# Autodesk Inventor assembly: vehicle assembly v2
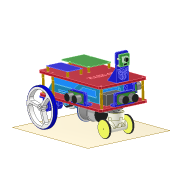
[picture p0: Inventor's stored thumbnail of the model, 180x180]
Saved by Autodesk Inventor 2022 (Build 260153000, 153)
## iProperties
Created: 2024-06-06
Part Number: vehicle assembly v2
Document SubType Name: Assembly
Designer: david
Author: david
## Documents named in this file (31)
- C:\Users\david\OneDrive\Documents\Inventor\WRO_FE_2024\vehicle assembly v2.iam
- C:\Users\david\OneDrive\Documents\Inventor\WRO_FE_2024\base plate.ipt
- C:\Users\david\OneDrive\Documents\Inventor\WRO_FE_2024\bearing holder.ipt
- C:\Users\david\OneDrive\Documents\Inventor\WRO_FE_2024\servo motor HS-7955TG.iam
- C:\Users\david\OneDrive\Documents\Inventor\WRO_FE_2024\steering.ipt
- C:\Users\david\OneDrive\Documents\Inventor\WRO_FE_2024\dfifferential.ipt
- C:\Users\david\OneDrive\Documents\Inventor\WRO_FE_2024\front wheel.ipt
- C:\Users\david\OneDrive\Documents\Inventor\WRO_FE_2024\driver gear.ipt
- C:\Users\david\OneDrive\Documents\Inventor\WRO_FE_2024\rear wheel 86mm.ipt
- C:\Users\david\OneDrive\Documents\Inventor\WRO_FE_2024\rear shaft v2.ipt
- rear shaft.ipt
- C:\Users\david\OneDrive\Documents\Inventor\WRO_FE_2024\12v DC motor mount.ipt
- C:\Users\david\OneDrive\Documents\Inventor\WRO_FE_2024\12v DC motor.ipt
- C:\Users\david\OneDrive\Documents\Inventor\WRO_FE_2024\driver gear adapter v2.ipt
- C:\Users\david\OneDrive\Documents\Inventor\WRO_FE_2024\stand M3-L10.ipt
- C:\Users\david\OneDrive\Documents\Inventor\WRO_FE_2024\top plate.ipt
- C:\Users\david\OneDrive\Documents\Inventor\WRO_FE_2024\raspberry pi.ipt
- C:\Users\david\OneDrive\Documents\Inventor\WRO_FE_2024\3s lipo battery.ipt
- C:\Users\david\OneDrive\Documents\Inventor\WRO_FE_2024\ultrasonic mount.ipt
- C:\Users\david\OneDrive\Documents\Inventor\WRO_FE_2024\US-015.ipt
- C:\Users\david\OneDrive\Documents\Inventor\WRO_FE_2024\stand M3-L30.ipt
- C:\Users\david\OneDrive\Documents\Inventor\WRO_FE_2024\LM2596 Buck Converter.ipt
- C:\Users\david\OneDrive\Documents\Inventor\WRO_FE_2024\camera mount.ipt
- C:\Users\david\OneDrive\Documents\Inventor\WRO_FE_2024\raspberry pi camera v2.ipt
- C:\Users\david\OneDrive\Documents\Inventor\WRO_FE_2024\stub.ipt
- C:\Users\david\OneDrive\Documents\Inventor\WRO_FE_2024\3S lipo holder.ipt
- C:\Users\david\OneDrive\Documents\Inventor\WRO_FE_2024\differential stopper.ipt
- C:\Users\david\OneDrive\Documents\Inventor\WRO_FE_2024\driver gear stopper.ipt
- C:\Users\david\OneDrive\Documents\Inventor\WRO_FE_2024\12v DC motor mount (3D printed).ipt
- C:\Users\david\OneDrive\Documents\Inventor\WRO_FE_2024\front shaft v3.ipt
- C:\Users\david\OneDrive\Documents\Inventor\WRO_FE_2024\steering bottom half.ipt
## Components (62 placed, 31 different names)
1. raspberry pi:2 — Insert:58, Insert:59
2. base plate:1 — Insert:60, Insert:61, Insert:62, Insert:63, Mate:9, Mate:10, Insert:72, Insert:73, Mate:11, Flush:6, Flush:7, Flush:8, Insert:74, Insert:75, Insert:128, Insert:129, Insert:130, Insert:131, Insert:132, Insert:133, Insert:134, Insert:135, Insert:136, Insert:137, Insert:138, Insert:139, Insert:140, Insert:141, Insert:144, Insert:145, Insert:154, Insert:155, Insert:156, Insert:157, Insert:158, Insert:159, Insert:160, Insert:161, Insert:162
3. top plate:1 — Insert:54, Insert:55, Insert:56, Insert:57, Insert:108, Insert:109, Insert:110, Insert:111, Insert:126, Insert:127, Insert:152, Insert:153
4. bearing holder:1 — Insert:138, Insert:139, Insert:142
5. bearing holder:2 — Insert:140, Insert:141
6. bearing holder:3 — Insert:136, Insert:137
7. bearing holder:4 — Insert:134, Insert:135, Insert:143
8. dfifferential:1
9. driver gear:1 — Insert:47
10. rear shaft v2: right — Insert:83, Angle:9, Insert:143
11. rear shaft v2: left — Insert:84, Angle:8, Insert:142
12. rear wheel 86mm: right — Insert:83, Angle:9
13. rear wheel 86mm: left — Tangent:1, Insert:84, Angle:8
14. 12v DC motor mount:1 — Insert:38, Insert:39, Insert:72, Insert:73
15. 12v DC motor:1 — Insert:38, Insert:39, Insert:46, Angle:5
16. driver gear adapter v2:1 — Insert:46, Insert:47, Angle:5
17. servo motor HS-7955TG:1 [sub-assembly] — Mate:2, Insert:20, Mate:9, Mate:10, Mate:11
18. steering:1 — Insert:20, Steering Angle, Insert:163, Insert:166, Insert:167
19. front wheel:1 — Insert:164, Angle:10
20. front wheel:2 — Insert:165, Angle:11
21. stand M3-L30:2 — Insert:60, Insert:150
22. stand M3-L30:3 — Insert:63, Insert:146
23. stand M3-L30:1 — Insert:61, Insert:151
24. stand M3-L30:4 — Insert:62, Insert:148
25. stand M3-L30:9 — Insert:74, Insert:149
26. stand M3-L30:10 — Insert:75, Insert:147
27. stand M3-L10:1 — Insert:55
28. stand M3-L10:2 — Insert:57
29. stand M3-L10:3 — Insert:54, Insert:59
30. stand M3-L10:4 — Insert:56, Insert:58
31. 3s lipo battery:1 — Mate:12, Mate:13, Flush:9
32. ultrasonic mount:1 — Insert:102, Insert:103, Insert:128, Insert:129
33. US-015:1 — Insert:102, Insert:103
34. ultrasonic mount:2 — Insert:104, Insert:105, Insert:130, Insert:131
35. ultrasonic mount:3 — Insert:106, Insert:107, Insert:132, Insert:133
36. US-015:2 — Insert:106, Insert:107
37. US-015:3 — Insert:104, Insert:105
38. LM2596 Buck Converter:1 — Insert:112, Insert:113
39. stand M3-L10:5 — Insert:109
40. stand M3-L10:6 — Insert:111
41. stand M3-L10:7 — Insert:108, Insert:112
42. stand M3-L10:8 — Insert:110, Insert:113
43. camera mount:1 — Insert:124, Insert:125, Insert:126, Insert:127
44. raspberry pi camera v2:1 — Insert:120, Insert:121, Insert:122, Insert:123
45. stub:1 — Insert:123
46. stub:2 — Insert:121, Insert:124
47. stub:3 — Insert:122
48. stub:4 — Insert:120, Insert:125
49. 3S lipo holder:1 — Insert:144, Insert:145, Mate:12, Mate:13
50. stand M3-L10:9 — Insert:148
51. stand M3-L10:10 — Insert:147
52. stand M3-L10:11 — Insert:151, Insert:153
53. stand M3-L10:12 — Insert:150
54. stand M3-L10:13 — Insert:149
55. stand M3-L10:14 — Insert:146, Insert:152
56. differential stopper:1
57. differential stopper:2 — Insert:157, Insert:158
58. differential stopper:3 — Insert:154, Insert:155, Insert:156
59. driver gear stopper:1 — Insert:159, Insert:160
60. 12v DC motor mount (3D printed):1 — Insert:161, Insert:162
61. rear shaft:5 — Insert:163, Insert:164, Angle:10, Insert:165, Angle:11
62. steering bottom half:1 — Insert:166, Insert:167
## Relationships (99: Insert 81, Angle 7, Mate 6, Flush 4, Tangent 1)
- Mate:2: servo motor HS-7955TG:1
- Insert:20: servo motor HS-7955TG:1 ↔ steering:1
- Steering Angle [Angle] (0 deg): steering:1
- Angle:4 (0 deg)
- Tangent:1: rear wheel 86mm: left
- Insert:38: 12v DC motor mount:1 ↔ 12v DC motor:1
- Insert:39: 12v DC motor mount:1 ↔ 12v DC motor:1
- Insert:46: 12v DC motor:1 ↔ driver gear adapter v2:1
- Insert:47: driver gear:1 ↔ driver gear adapter v2:1
- Angle:5 (180 deg): 12v DC motor:1 ↔ driver gear adapter v2:1
- Insert:54: top plate:1 ↔ stand M3-L10:3
- Insert:55: top plate:1 ↔ stand M3-L10:1
- Insert:56: top plate:1 ↔ stand M3-L10:4
- Insert:57: top plate:1 ↔ stand M3-L10:2
- Insert:58: raspberry pi:2 ↔ stand M3-L10:4
- Insert:59: raspberry pi:2 ↔ stand M3-L10:3
- Insert:60: base plate:1 ↔ stand M3-L30:2
- Insert:61: base plate:1 ↔ stand M3-L30:1
- Insert:62: base plate:1 ↔ stand M3-L30:4
- Insert:63: base plate:1 ↔ stand M3-L30:3
- Mate:9: base plate:1 ↔ servo motor HS-7955TG:1
- Mate:10: base plate:1 ↔ servo motor HS-7955TG:1
- Insert:72: base plate:1 ↔ 12v DC motor mount:1
- Insert:73: base plate:1 ↔ 12v DC motor mount:1
- Mate:11: base plate:1 ↔ servo motor HS-7955TG:1
- Flush:6: base plate:1
- Flush:7: base plate:1
- Flush:8: base plate:1
- Insert:74: base plate:1 ↔ stand M3-L30:9
- Insert:75: base plate:1 ↔ stand M3-L30:10
- Insert:83: rear shaft v2: right ↔ rear wheel 86mm: right
- Insert:84: rear shaft v2: left ↔ rear wheel 86mm: left
- Angle:8 (180 deg): rear shaft v2: left ↔ rear wheel 86mm: left
- Angle:9 (180 deg): rear shaft v2: right ↔ rear wheel 86mm: right
- Insert:102: ultrasonic mount:1 ↔ US-015:1
- Insert:103: ultrasonic mount:1 ↔ US-015:1
- Insert:104: ultrasonic mount:2 ↔ US-015:3
- Insert:105: ultrasonic mount:2 ↔ US-015:3
- Insert:106: ultrasonic mount:3 ↔ US-015:2
- Insert:107: ultrasonic mount:3 ↔ US-015:2
- Insert:108: top plate:1 ↔ stand M3-L10:7
- Insert:109: top plate:1 ↔ stand M3-L10:5
- Insert:110: top plate:1 ↔ stand M3-L10:8
- Insert:111: top plate:1 ↔ stand M3-L10:6
- Insert:112: LM2596 Buck Converter:1 ↔ stand M3-L10:7
- Insert:113: LM2596 Buck Converter:1 ↔ stand M3-L10:8
- Insert:120: raspberry pi camera v2:1 ↔ stub:4
- Insert:121: raspberry pi camera v2:1 ↔ stub:2
- Insert:122: raspberry pi camera v2:1 ↔ stub:3
- Insert:123: raspberry pi camera v2:1 ↔ stub:1
- Insert:124: camera mount:1 ↔ stub:2
- Insert:125: camera mount:1 ↔ stub:4
- Insert:126: top plate:1 ↔ camera mount:1
- Insert:127: top plate:1 ↔ camera mount:1
- Insert:128: base plate:1 ↔ ultrasonic mount:1
- Insert:129: base plate:1 ↔ ultrasonic mount:1
- Insert:130: base plate:1 ↔ ultrasonic mount:2
- Insert:131: base plate:1 ↔ ultrasonic mount:2
- Insert:132: base plate:1 ↔ ultrasonic mount:3
- Insert:133: base plate:1 ↔ ultrasonic mount:3
- Insert:134: base plate:1 ↔ bearing holder:4
- Insert:135: base plate:1 ↔ bearing holder:4
- Insert:136: base plate:1 ↔ bearing holder:3
- Insert:137: base plate:1 ↔ bearing holder:3
- Insert:138: base plate:1 ↔ bearing holder:1
- Insert:139: base plate:1 ↔ bearing holder:1
- Insert:140: base plate:1 ↔ bearing holder:2
- Insert:141: base plate:1 ↔ bearing holder:2
- Insert:142: bearing holder:1 ↔ rear shaft v2: left
- Insert:143: bearing holder:4 ↔ rear shaft v2: right
- Insert:144: base plate:1 ↔ 3S lipo holder:1
- Insert:145: base plate:1 ↔ 3S lipo holder:1
- Mate:12: 3s lipo battery:1 ↔ 3S lipo holder:1
- Mate:13: 3s lipo battery:1 ↔ 3S lipo holder:1
- Insert:146: stand M3-L30:3 ↔ stand M3-L10:14
- Insert:147: stand M3-L30:10 ↔ stand M3-L10:10
- Insert:148: stand M3-L30:4 ↔ stand M3-L10:9
- Insert:149: stand M3-L30:9 ↔ stand M3-L10:13
- Insert:150: stand M3-L30:2 ↔ stand M3-L10:12
- Insert:151: stand M3-L30:1 ↔ stand M3-L10:11
- Insert:152: top plate:1 ↔ stand M3-L10:14
- Insert:153: top plate:1 ↔ stand M3-L10:11
- Flush:9: 3s lipo battery:1
- Insert:154: base plate:1 ↔ differential stopper:3
- Insert:155: base plate:1 ↔ differential stopper:3
- Insert:156: base plate:1 ↔ differential stopper:3
- Insert:157: base plate:1 ↔ differential stopper:2
- Insert:158: base plate:1 ↔ differential stopper:2
- Insert:159: base plate:1 ↔ driver gear stopper:1
- Insert:160: base plate:1 ↔ driver gear stopper:1
- Insert:161: base plate:1 ↔ 12v DC motor mount (3D printed):1
- Insert:162: base plate:1 ↔ 12v DC motor mount (3D printed):1
- Insert:163: steering:1 ↔ rear shaft:5
- Insert:164: front wheel:1 ↔ rear shaft:5
- Angle:10 (0 deg): front wheel:1 ↔ rear shaft:5
- Insert:165: front wheel:2 ↔ rear shaft:5
- Angle:11 (0 deg): front wheel:2 ↔ rear shaft:5
- Insert:166: steering:1 ↔ steering bottom half:1
- Insert:167: steering:1 ↔ steering bottom half:1
